# Autodesk Inventor assembly: Base2
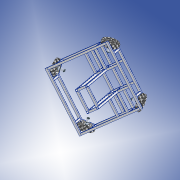
[picture p0: Inventor's stored thumbnail of the model, 180x180]
Saved by Autodesk Inventor 2017 (Build 210142000, 142)
## iProperties
Created: 2017-06-13
Part Number: Base2
Document SubType Name: Assembly
Designer: zallen
Author: zallen
## Documents named in this file (4)
- C:\Users\zallen\Documents\GitHub\cr-laundry-robot\src\Base 2\Base2.iam
- C:\Users\zallen\Documents\GitHub\cr-laundry-robot\src\Base 2\Chassis\Chassis.iam
- C:\Users\zallen\Documents\GitHub\cr-laundry-robot\lib\DC Motor with Encoder\Motor.ipt
- C:\Users\zallen\Documents\GitHub\cr-laundry-robot\lib\Omni Wheel 6in\217-2585.ipt
## Components (9 placed, 3 different names)
1. Chassis:1 [sub-assembly] — Mate:1, Mate:2, Mate:3, Mate:4, Mate:5, Mate:6, Mate:7, Mate:8, Mate:10, Mate:12, Mate:14, Mate:16
2. Motor:1 — Mate:1, Mate:2, Mate:13
3. Motor:2 — Mate:7, Mate:8, Mate:9
4. Motor:3 — Mate:5, Mate:6, Mate:15
5. Motor:4 — Mate:3, Mate:4, Mate:11
6. 217-2585:1 — Mate:9, Mate:10
7. 217-2585:2 — Mate:11, Mate:12
8. 217-2585:3 — Mate:13, Mate:14
9. 217-2585:4 — Mate:15, Mate:16
## Relationships (16: Mate 16)
- Mate:1: Chassis:1 ↔ Motor:1
- Mate:2: Chassis:1 ↔ Motor:1
- Mate:3: Chassis:1 ↔ Motor:4
- Mate:4: Chassis:1 ↔ Motor:4
- Mate:5: Chassis:1 ↔ Motor:3
- Mate:6: Chassis:1 ↔ Motor:3
- Mate:7: Chassis:1 ↔ Motor:2
- Mate:8: Chassis:1 ↔ Motor:2
- Mate:9: Motor:2 ↔ 217-2585:1
- Mate:10: Chassis:1 ↔ 217-2585:1
- Mate:11: Motor:4 ↔ 217-2585:2
- Mate:12: Chassis:1 ↔ 217-2585:2
- Mate:13: Motor:1 ↔ 217-2585:3
- Mate:14: Chassis:1 ↔ 217-2585:3
- Mate:15: Motor:3 ↔ 217-2585:4
- Mate:16: Chassis:1 ↔ 217-2585:4
